# Autodesk Inventor assembly: liarAssembly
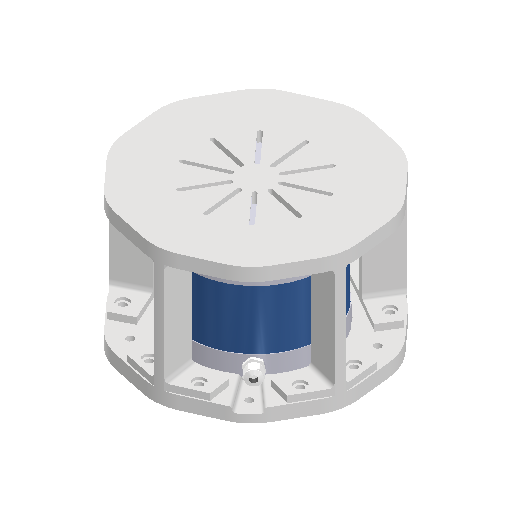
[picture p0: Inventor's stored thumbnail of the model, 512x512]
Saved by Autodesk Inventor 2025 (Build 290162000, 162)
## iProperties
Created: 2024-12-09
Part Number: liarAssembly
Document SubType Name: Assembly
Designer: derm
Author: derm
## Documents named in this file (5)
- C:\Users\derm\Desktop\puppycat\liarAssembly.iam
- C:\Users\derm\Desktop\puppycat\86-0138 REV 2, ENVELOPE, VLP-32C M12M\86-0138 REV 2, ENVELOPE, VLP-32C M12M.ipt
- C:\Users\derm\Desktop\puppycat\lidarCage.ipt
- C:\Users\derm\Desktop\puppycat\lidarCageTop.ipt
- C:\Users\derm\Desktop\puppycat\lidarFOV.ipt
## Components (4 placed, 4 different names)
1. 86-0138 REV 2, ENVELOPE, VLP-32C M12M:1 — Mate:4, Mate:5, Mate:6
2. lidarCage:1 — Flush:1, Flush:2, Flush:3
3. lidarCageTop:1 — Flush:1, Flush:2, Flush:3
4. lidarFOV:1 — Mate:4, Mate:5, Mate:6
## Relationships (8: Mate 5, Flush 3)
- [Mate]: 86-0138 REV 2, ENVELOPE, VLP-32C M12M:1 ↔ lidarCage:1
- [Mate]: 86-0138 REV 2, ENVELOPE, VLP-32C M12M:1 ↔ lidarCage:1
- Flush:1: lidarCage:1 ↔ lidarCageTop:1
- Mate:4: 86-0138 REV 2, ENVELOPE, VLP-32C M12M:1 ↔ lidarFOV:1
- Mate:5: 86-0138 REV 2, ENVELOPE, VLP-32C M12M:1 ↔ lidarFOV:1
- Mate:6: 86-0138 REV 2, ENVELOPE, VLP-32C M12M:1 ↔ lidarFOV:1
- Flush:2: lidarCage:1 ↔ lidarCageTop:1
- Flush:3: lidarCage:1 ↔ lidarCageTop:1
